# Autodesk Inventor assembly: Link_Shim
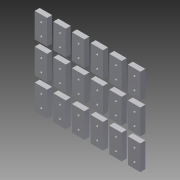
[picture p0: Inventor's stored thumbnail of the model, 180x180]
Saved by Autodesk Inventor 2013 (Build 170138000, 138)
## iProperties
Created: 2014-04-21
Part Number: Link_Shim
Document SubType Name: Assembly
Designer: andou
Author: andou
## Documents named in this file (2)
- C:\Users\andou\Documents\GitHub\Robotics-Project\design\RoboticsProject\project_4\cnc_data\Link_Shim_16.iam
- C:\Users\andou\Documents\GitHub\Robotics-Project\design\RoboticsProject\project_4\cnc_data\Leg_Link_Shim.ipt
## Components (18 placed, 1 different names)
1. Leg_Link_Shim:1
2. Leg_Link_Shim:2
3. Leg_Link_Shim:3
4. Leg_Link_Shim:4
5. Leg_Link_Shim:5
6. Leg_Link_Shim:6
7. Leg_Link_Shim:7
8. Leg_Link_Shim:8
9. Leg_Link_Shim:9
10. Leg_Link_Shim:10
11. Leg_Link_Shim:11
12. Leg_Link_Shim:12
13. Leg_Link_Shim:13
14. Leg_Link_Shim:14
15. Leg_Link_Shim:15
16. Leg_Link_Shim:16
17. Leg_Link_Shim:17
18. Leg_Link_Shim:18
## Component patterns: (18 elements, first: Leg_Link_Shim:1)
